# Autodesk Inventor assembly: componentes
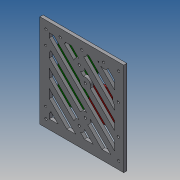
[picture p0: Inventor's stored thumbnail of the model, 180x180]
Saved by Autodesk Inventor 2017 (Build 210142000, 142)
## iProperties
Part Number: componentes
Material: Genérico
Document SubType Name: Assembly
Designer: FABLAB
Author: FABLAB
## Documents named in this file (4)
- C:\Users\Leo\Documents\GitHub\actor-re-actor\models\inventor-caja\Piezas\componentes.iam
- C:\Users\Leo\Documents\GitHub\actor-re-actor\models\inventor-caja\Case\bandeja componentes.ipt
- C:\Users\Leo\Documents\GitHub\actor-re-actor\models\inventor-caja\Piezas\driver motor.ipt
- C:\Users\Leo\Documents\GitHub\actor-re-actor\models\inventor-caja\Piezas\dimmer.ipt
## Components (3 placed, 3 different names)
1. bandeja componentes:1 — Coincidencia:1, Nivelación:1, Coincidencia:3
2. driver motor:1 — Coincidencia:1, Nivelación:1, Nivelación:2, Coincidencia:2, Nivelación:3
3. dimmer:1 — Coincidencia:2, Nivelación:3, Coincidencia:3
## Relationships (6: Mate 3, Flush 3)
- Coincidencia:1 [Mate] (15 mm): bandeja componentes:1 ↔ driver motor:1
- Nivelación:1 [Flush] (4 mm): bandeja componentes:1 ↔ driver motor:1
- Nivelación:2 [Flush] (3 mm): driver motor:1
- Coincidencia:2 [Mate] (2 mm): driver motor:1 ↔ dimmer:1
- Nivelación:3 [Flush] (14 mm): driver motor:1 ↔ dimmer:1
- Coincidencia:3 [Mate] (3 mm): bandeja componentes:1 ↔ dimmer:1
